# Autodesk Inventor assembly: bed
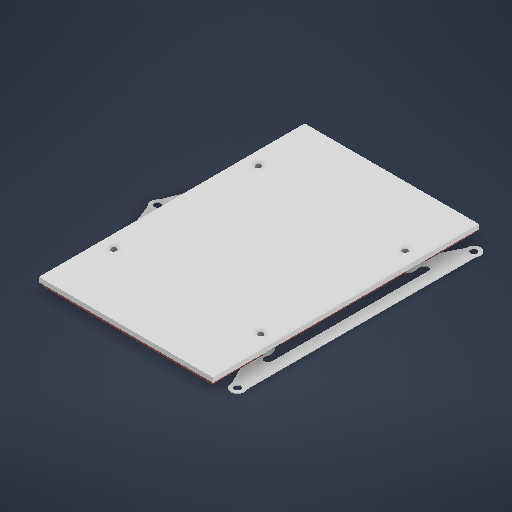
[picture p0: Inventor's stored thumbnail of the model, 512x512]
Saved by Autodesk Inventor 2025 (Build 290162000, 162)
## iProperties
Created: 2024-06-24
Part Number: bed
Document SubType Name: Assembly
Designer: Windows 7 was better
Author: Windows 7 was better
## Documents named in this file (4)
- C:\Users\Windows 7 was better\Documents\ReplicatorPlusConversion\CAD\bed-oops.iam
- C:\Users\Windows 7 was better\Documents\ReplicatorPlusConversion\CAD\heater-oops.ipt
- C:\Users\Windows 7 was better\Documents\ReplicatorPlusConversion\CAD\bed-oops.ipt
- C:\Users\Windows 7 was better\Documents\ReplicatorPlusConversion\CAD\bed-plate_oops.ipt
## Components (3 placed, 3 different names)
1. heater-oops:1 — Flush:1
2. bed-oops:1
3. bed-plate_oops:1 — Flush:1
## Relationships (1: Flush 1)
- Flush:1: heater-oops:1 ↔ bed-plate_oops:1
